# Autodesk Inventor assembly: pryBar
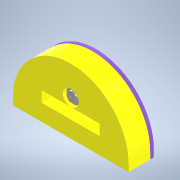
[picture p0: Inventor's stored thumbnail of the model, 180x180]
Saved by Autodesk Inventor 2021.1 (Build 251245000, 245)
## iProperties
Created: 2020-09-14
Part Number: pryBar
Document SubType Name: Assembly
Designer: robst
Author: robst
## Documents named in this file (6)
- C:\git\CAD-Development\robSteele\ShapeWays\ToolBelt\pryBar.iam
- C:\git\CAD-Development\robSteele\ShapeWays\ToolBelt\dRingHolder.ipt
- C:\git\CAD-Development\robSteele\ShapeWays\ToolBelt\dRingHolderBottom.ipt
- C:\Users\robst\Documents\Inventor\Content Center Files\R2021\en-US\ANSI B18.22.1\ANSI B18.22.1 - No. 10 - Type A.ipt
- C:\Users\robst\Documents\Inventor\Content Center Files\R2021\en-US\U UNC 2605\Unbrako - 10 x 7_8 - 24(10).ipt
- C:\Users\robst\Documents\Inventor\Content Center Files\R2021\en-US\ANSI B 18.2.2(2)\ANSI B 18.2.2 - #10-24(2).ipt
## Components (6 placed, 5 different names)
1. dRingHolder:1 — Mate:1, Mate:2, Mate:3, Mate:4, Mate:5
2. dRingHolderBottom:1 — Mate:1, Mate:2, Mate:6
3. Plain Washer (Inch) No. 10 - Type A:1 — Mate:3, Mate:4, Insert:1
4. Unbrako UNC Hex Socket Button Cap - Inch 10 x 7/8:1 — Insert:1
5. Plain Washer (Inch) No. 10 - Type A:2 — Mate:5, Mate:6, Insert:2
6. Low Crown #10-24:1 — Insert:2
## Relationships (8: Mate 6, Insert 2)
- Mate:1: dRingHolder:1 ↔ dRingHolderBottom:1
- Mate:2: dRingHolder:1 ↔ dRingHolderBottom:1
- Mate:3: dRingHolder:1 ↔ Plain Washer (Inch) No. 10 - Type A:1
- Mate:4: dRingHolder:1 ↔ Plain Washer (Inch) No. 10 - Type A:1
- Insert:1: Plain Washer (Inch) No. 10 - Type A:1 ↔ Unbrako UNC Hex Socket Button Cap - Inch 10 x 7/8:1
- Mate:5: dRingHolder:1 ↔ Plain Washer (Inch) No. 10 - Type A:2
- Mate:6: dRingHolderBottom:1 ↔ Plain Washer (Inch) No. 10 - Type A:2
- Insert:2: Plain Washer (Inch) No. 10 - Type A:2 ↔ Low Crown #10-24:1
